# Autodesk Inventor assembly: CircuitBoardV2
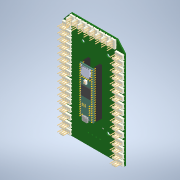
[picture p0: Inventor's stored thumbnail of the model, 180x180]
Saved by Autodesk Inventor 2021 (Build 250183000, 183)
## iProperties
Company: A Company
Created: 2021-03-17
Part Number: CircuitBoardV2
Description: KiCad electronic assembly
Document SubType Name: Assembly
Designer: Collin
Authority: Unknown
Title: CircuitBoardV2.step
Author: An Author
Sending System: KiCad to STEP converter
Preprocessor: Open CASCADE STEP processor 6.9
## Documents named in this file (6)
- H:\Projects\RGB Controller\Teensy-PC_RGB_Controller\2 PCB\CAD\V2\CircuitBoardV2.iam
- H:\Projects\RGB Controller\Teensy-PC_RGB_Controller\2 PCB\CAD\V2\R_0603_1608Metric.iam
- H:\Projects\RGB Controller\Teensy-PC_RGB_Controller\2 PCB\CAD\V2\FanPinHeader_1x04_P2.54mm_Vertical.iam
- H:\Projects\RGB Controller\Teensy-PC_RGB_Controller\2 PCB\CAD\V2\PinSocket_1x24_P2.54mm_Vertical.iam
- H:\Projects\RGB Controller\Teensy-PC_RGB_Controller\2 PCB\CAD\V2\COMPOUND.ipt
- H:\Projects\RGB Controller\Teensy-PC_RGB_Controller\2 PCB\CAD\teensy-4-1-development-board-1.snapshot.5\Teensy 4.1 (With Headers).iam
## Components (45 placed, 45 different names)
1. 2 [sub-assembly]
2. 4 [sub-assembly]
3. 5 [sub-assembly]
4. 6 [sub-assembly]
5. 7 [sub-assembly]
6. 8 [sub-assembly]
7. 9 [sub-assembly]
8. 10 [sub-assembly]
9. 11 [sub-assembly]
10. 12 [sub-assembly]
11. 13 [sub-assembly]
12. 14 [sub-assembly]
13. 15 [sub-assembly]
14. 16 [sub-assembly]
15. 17 [sub-assembly]
16. 18 [sub-assembly]
17. 19 [sub-assembly]
18. 20 [sub-assembly]
19. 21 [sub-assembly]
20. 22 [sub-assembly]
21. 23 [sub-assembly]
22. 25 [sub-assembly]
23. 26 [sub-assembly] — Mate:1, Mate:2, Mate:3
24. 27 [sub-assembly]
25. 28 [sub-assembly]
26. 29 [sub-assembly]
27. 30 [sub-assembly]
28. 31 [sub-assembly]
29. 32 [sub-assembly]
30. 33 [sub-assembly]
31. 34 [sub-assembly]
32. 35 [sub-assembly]
33. 36 [sub-assembly]
34. 37 [sub-assembly]
35. 38 [sub-assembly]
36. 39 [sub-assembly]
37. 40 [sub-assembly]
38. 41 [sub-assembly]
39. 42 [sub-assembly]
40. 43 [sub-assembly]
41. 44 [sub-assembly]
42. 45 [sub-assembly]
43. 46 [sub-assembly]
44. 47
45. Teensy 4.1 (With Headers):1 [sub-assembly] — Mate:1, Mate:2, Mate:3
## Relationships (3: Mate 3)
- Mate:1: 26 ↔ Teensy 4.1 (With Headers):1
- Mate:2: 26 ↔ Teensy 4.1 (With Headers):1
- Mate:3: 26 ↔ Teensy 4.1 (With Headers):1
